# Autodesk Inventor assembly: Shock Strut
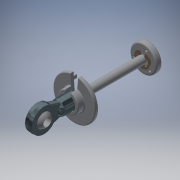
[picture p0: Inventor's stored thumbnail of the model, 180x180]
Saved by Autodesk Inventor 2019 (Build 230136000, 136)
## iProperties
Created: 2019-12-01
Part Number: Shock Strut
Document SubType Name: Assembly
Designer: Jopa
Author: Jopa
## Documents named in this file (6)
- C:\Users\Jopa\Desktop\Suspension\Shock Strut.iam
- C:\Users\Jopa\Desktop\Suspension\Shock Shaft.ipt
- C:\Users\Jopa\Desktop\Suspension\Piston of Suspension.ipt
- C:\Users\Jopa\Desktop\Suspension\E-Clip.ipt
- C:\Users\Jopa\Desktop\Suspension\Ball End.iam
- C:\Users\Jopa\Desktop\Suspension\Spring Cup.ipt
## Components (6 placed, 5 different names)
1. Shock Shaft:1 — Mate:1, Flush:1, Mate:6, Mate:7, Mate:9
2. Piston of Suspension:1 — Mate:1, Mate:2, Mate:3, Mate:4, Mate:5, Flush:1
3. E-Clip:1 — Mate:4, Mate:5
4. E-Clip:2 — Mate:2, Mate:3
5. Ball End:1 [sub-assembly] — Mate:6, Mate:7, Mate:8
6. Spring Cup:1 — Mate:8, Mate:9
## Relationships (10: Mate 9, Flush 1)
- Mate:1: Shock Shaft:1 ↔ Piston of Suspension:1
- Mate:2: Piston of Suspension:1 ↔ E-Clip:2
- Mate:3: Piston of Suspension:1 ↔ E-Clip:2
- Mate:4: Piston of Suspension:1 ↔ E-Clip:1
- Mate:5: Piston of Suspension:1 ↔ E-Clip:1
- Flush:1: Shock Shaft:1 ↔ Piston of Suspension:1
- Mate:6: Shock Shaft:1 ↔ Ball End:1
- Mate:7: Shock Shaft:1 ↔ Ball End:1
- Mate:8: Ball End:1 ↔ Spring Cup:1
- Mate:9: Shock Shaft:1 ↔ Spring Cup:1
